# Autodesk Inventor assembly: MG_996R v1
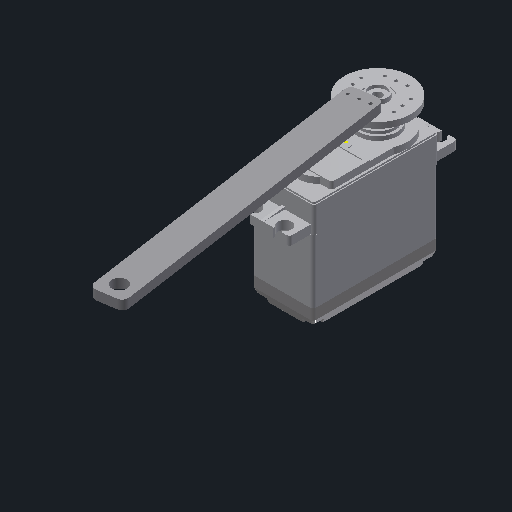
[picture p0: Inventor's stored thumbnail of the model, 512x512]
Saved by Autodesk Inventor 2023.6 (Build 276521000, 521)
## iProperties
Created: 2016-09-26
Part Number: MG_996R v1
Document SubType Name: Assembly
Designer: Julian
Author: Julian
## Documents named in this file (7)
- C:\Users\user\Downloads\servo-mg996r-1.snapshot.11\MG_996R v1.iam
- C:\Users\user\Downloads\servo-mg996r-1.snapshot.11\Base.ipt
- C:\Users\user\Downloads\servo-mg996r-1.snapshot.11\Medio.ipt
- C:\Users\user\Downloads\servo-mg996r-1.snapshot.11\Top.ipt
- C:\Users\user\Downloads\servo-mg996r-1.snapshot.11\Eje.ipt
- C:\Users\user\Downloads\servo-mg996r-1.snapshot.11\Acople circular.ipt
- C:\Users\user\OneDrive\Documents\FP V2 Servo Arm v2.ipt
## Components (6 placed, 6 different names)
1. Top:1 — Rígido:2, De rotación:1
2. Medio:1 — Rígido:1, Rígido:2
3. Base:1 — Rígido:1
4. Eje:1 — De rotación:1, Mate:1, Mate:2
5. Acople circular:1 — Mate:1, Mate:2, Mate:3, Mate:4, Mate:5
6. FP V2 Servo Arm v2:1 — Mate:3, Mate:4, Mate:5
## Relationships (8: Mate 5, WeldJoint 2, RevoluteJoint 1)
- Rígido:1 [WeldJoint]: Medio:1 ↔ Base:1
- Rígido:2 [WeldJoint]: Top:1 ↔ Medio:1
- De rotación:1 [RevoluteJoint]: Top:1 ↔ Eje:1
- Mate:1: Eje:1 ↔ Acople circular:1
- Mate:2: Eje:1 ↔ Acople circular:1
- Mate:3: Acople circular:1 ↔ FP V2 Servo Arm v2:1
- Mate:4: Acople circular:1 ↔ FP V2 Servo Arm v2:1
- Mate:5: Acople circular:1 ↔ FP V2 Servo Arm v2:1
